# Autodesk Inventor assembly: ellensuly
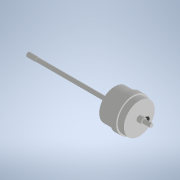
[picture p0: Inventor's stored thumbnail of the model, 180x180]
Saved by Autodesk Inventor 2021.4 (Build 254397000, 397)
## iProperties
Created: 2023-12-03
Part Number: ellensuly
Document SubType Name: Assembly
Designer: vtoth
Author: vtoth
## Documents named in this file (4)
- C:\Users\vtoth\OneDrive - Budapesti Műszaki és Gazdaságtudományi Egyetem\5_felev\CAD\hf2_v2\ellensuly.iam
- C:\Users\vtoth\OneDrive - Budapesti Műszaki és Gazdaságtudományi Egyetem\5_felev\CAD\hf2_v2\ellensuly_rud.ipt
- C:\Users\vtoth\OneDrive - Budapesti Műszaki és Gazdaságtudományi Egyetem\5_felev\CAD\hf2_v2\ellensuly_suly.ipt
- C:\Users\vtoth\OneDrive - Budapesti Műszaki és Gazdaságtudományi Egyetem\5_felev\CAD\hf2_v2\ContentCenter\en-US\ISO 4018\ISO 4018 - M6 x 12.ipt
## Components (3 placed, 3 different names)
1. ellensuly_rud:1 — Tangent:1, Mate:2, Mate:3, Flush:1
2. ellensuly_suly:1 — Mate:1, Angle:1, Mate:2, Mate:3, Flush:1
3. ISO 4018 M6 x 12:1 — Mate:1, Tangent:1, Angle:1
## Relationships (6: Mate 3, Tangent 1, Angle 1, Flush 1)
- Mate:1: ellensuly_suly:1 ↔ ISO 4018 M6 x 12:1
- Tangent:1: ellensuly_rud:1 ↔ ISO 4018 M6 x 12:1
- Angle:1 (0 deg): ellensuly_suly:1 ↔ ISO 4018 M6 x 12:1
- Mate:2: ellensuly_rud:1 ↔ ellensuly_suly:1
- Mate:3: ellensuly_rud:1 ↔ ellensuly_suly:1
- Flush:1 (-40 mm): ellensuly_rud:1 ↔ ellensuly_suly:1
